# Autodesk Inventor assembly: WANYOIKE
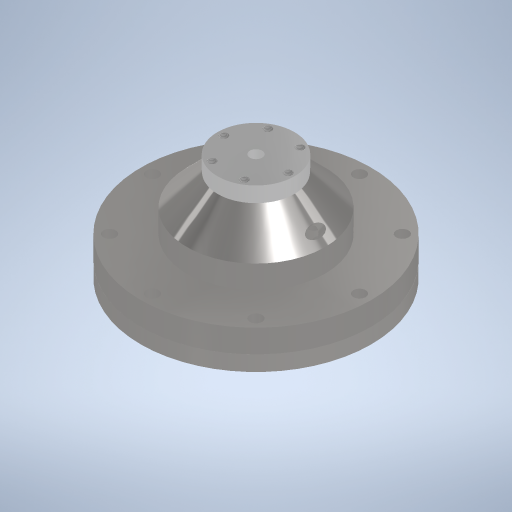
[picture p0: Inventor's stored thumbnail of the model, 512x512]
Saved by Autodesk Inventor 2023 (Build 270158000, 158)
## iProperties
Created: 2022-09-20
Part Number: WANYOIKE
Document SubType Name: Assembly
Designer: pc
Author: pc
## Documents named in this file (6)
- C:\Users\station\Documents\Project\Liquid-engine-cooling-system\design files\injector_design_files\WANYOIKE.iam
- C:\Users\station\Documents\Project\Liquid-engine-cooling-system\design files\injector_design_files\final injector body.ipt
- C:\Users\station\Documents\Project\Liquid-engine-cooling-system\design files\injector_design_files\Orifice Plate.ipt
- C:\Users\station\Documents\Project\Liquid-engine-cooling-system\design files\injector_design_files\Pintle tip vip.ipt
- C:\Users\station\Documents\Project\Liquid-engine-cooling-system\design files\injector_design_files\pintle body.ipt
- C:\Users\station\Documents\Project\Liquid-engine-cooling-system\design files\injector_design_files\faceplate.ipt
## Components (5 placed, 5 different names)
1. final injector body:1 — Mate:1, Rotational:1, Mate:2, Rotational:2, Mate:3, Mate:6, Mate:7
2. Pintle tip vip:1 — Mate:3, Rotational:3, Mate:4
3. pintle body:1 — Mate:2, Rotational:2, Rotational:3
4. faceplate:1 — Mate:4, Mate:6, Mate:7
5. Orifice Plate:1 — Mate:1, Rotational:1
## Relationships (9: Mate 6, RevoluteJoint 3)
- Mate:1: final injector body:1 ↔ Orifice Plate:1
- Rotational:1 [RevoluteJoint]: final injector body:1 ↔ Orifice Plate:1
- Mate:2: final injector body:1 ↔ pintle body:1
- Rotational:2 [RevoluteJoint]: final injector body:1 ↔ pintle body:1
- Mate:3: final injector body:1 ↔ Pintle tip vip:1
- Rotational:3 [RevoluteJoint]: Pintle tip vip:1 ↔ pintle body:1
- Mate:4: Pintle tip vip:1 ↔ faceplate:1
- Mate:6: final injector body:1 ↔ faceplate:1
- Mate:7: final injector body:1 ↔ faceplate:1
